# Autodesk Inventor assembly: Ensamble sin tapa + rodamientos
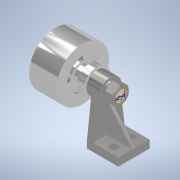
[picture p0: Inventor's stored thumbnail of the model, 180x180]
Saved by Autodesk Inventor 2021 (Build 250183000, 183)
## iProperties
Created: 2021-01-10
Part Number: Ensamble sin tapa + rodamientos
Document SubType Name: Assembly
Designer: dieku
Author: dieku
## Documents named in this file (3)
- C:\Users\dieku\Documents\GitHub\tallerDibujoIngenieria\Ensambles\Ensamble sin tapa + rodamientos.iam
- C:\Users\dieku\Documents\GitHub\tallerDibujoIngenieria\Ensambles\Ensamble eje + chaveta.iam
- C:\Users\dieku\Documents\GitHub\tallerDibujoIngenieria\Ensambles\Rodamiento doble + arandela + cilindro separador.iam
## Components (2 placed, 2 different names)
1. Ensamble eje + chaveta:1 [sub-assembly] — Insert:1
2. Rodamiento doble + arandela + cilindro separador:1 [sub-assembly] — Insert:1
## Relationships (1: Insert 1)
- Insert:1: Ensamble eje + chaveta:1 ↔ Rodamiento doble + arandela + cilindro separador:1
